# Autodesk Inventor assembly: Ensamblaje1
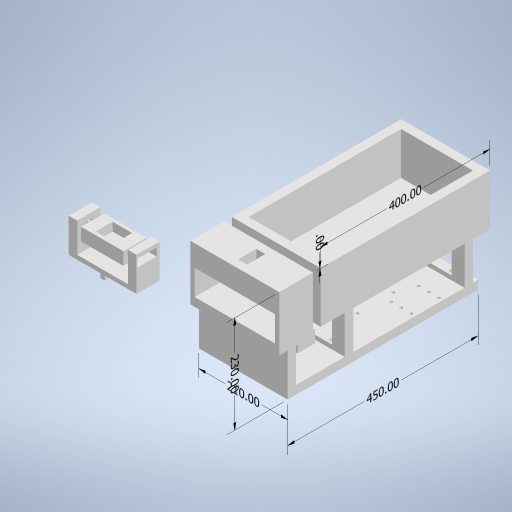
[picture p0: Inventor's stored thumbnail of the model, 512x512]
Saved by Autodesk Inventor 2023 (Build 270158000, 158)
## iProperties
Created: 2022-07-04
Part Number: Ensamblaje1
Document SubType Name: Assembly
Designer: inigo
Author: inigo
## Documents named in this file (6)
- D:\projects\FoBo\model\Ensamblaje1.iam
- D:\projects\FoBo\model\base.ipt
- D:\projects\FoBo\model\camera_support.ipt
- D:\projects\FoBo\model\camera_support_2.ipt
- D:\projects\FoBo\model\camera_support_union.ipt
- D:\projects\FoBo\model\container.ipt
## Components (5 placed, 5 different names)
1. base:1 — Coincidencia:2, Coincidencia:3
2. camera_support:1
3. camera_support_2:1 — Coincidencia:1
4. camera_support_union:1 — Coincidencia:1
5. container:1 — Coincidencia:2, Coincidencia:3
## Relationships (3: Mate 3)
- Coincidencia:1 [Mate]: camera_support_2:1 ↔ camera_support_union:1
- Coincidencia:2 [Mate]: base:1 ↔ container:1
- Coincidencia:3 [Mate]: base:1 ↔ container:1
